# Autodesk Inventor assembly: 536206 ADN-12-15-A-P-A---(asm_0)
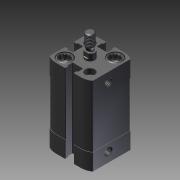
[picture p0: Inventor's stored thumbnail of the model, 180x180]
Saved by Autodesk Inventor 2011 SP1 (Build 150282100, 282)
## iProperties
Created: 2018-05-28
Part Number: 536206 ADN-12-15-A-P-A---(asm_0)
Catalog Web Link: www.cadenas.de
Description: ADN-Compact cylinder
Vendor: FESTO
Document SubType Name: Assembly
Designer: psAdmin
Manufacturer: FESTO
Mass: 95 g
Category: PARTsolutions
Company: FESTO
Title: 536206 ADN-12-15-A-P-A
Author: Cadenas PARTsolutions
Comments: Compact cylinder
PSOL_IDENT_0: {$CADENAS_DATA\23d-libs\festo\parts\a\adn\adn_std_tab.prj},213 {VTYP=3D},{STYP=ASSTAB},{NB=536206 AD
PSOL_IDENT_1: N-12-15-A-P-A---(asm_0)},{LINA=536206 ADN-12-15-A-P-A},{NN=ADN},{DATE=17.05.2018 10:40:18},{GEOMDATE=
PSOL_IDENT_2: 24.04.2017 11:47:47},{VERSION=},{LINEID=140},{LINESUBID=-1},{WBVAR=HUBST}  {NB=536206 ADN-12-15-A-P-
PSOL_IDENT_3: A---(asm_0)},{LINA=536206 ADN-12-15-A-P-A},{KT=DUMMY},{TNR=536206},{TYP=ADN-12-15-A-P-A},{KDM=12},{H
PSOL_IDENT_4: UB=15},{HUBST=0},{DF=P},{TH=A},{Q=0},{S2=0},{K2=0},{K5=0},{K8=0},{ZZ=0},{A=10.000},{AF=8.000},{BG=17
PSOL_IDENT_5: .000},{D1=9.000},{D5=6.000},{E=27.500},{EE=M5},{EEN=5.000},{EEK=4.019},{G=10.500},{KF=M3},{KFN=3.000
PSOL_IDENT_6: },{KFK=2.459},{KFNW=3},{KFKW=2.459},{KK=M5},{KKN=5.000},{KKK=4.019},{KKNW=5},{KKKW=4.019},{L3=3.500}
PSOL_IDENT_7: ,{L12=2.700},{MM=6.000},{PL=6.000},{RR=3.200},{RT=M4},{RTN=4.000},{RTK=3.242},{SW=5.000},{T1=2.100},
PSOL_IDENT_8: {T4=1.500},{TG=16.000},{WH=4.200},{ZA=35.000},{ZB=39.200},{J3=2.000},{SWQ=5.000},{RA=0.000},{RU=16.6
PSOL_IDENT_9: 00},{RT1=3.400},{RB1=5.400},{RB2=6.800},{R1=10.350},{R2=0.600},{FORM=1},{MASSBKS=0.009},{MASSHKS=0.0
PSOL_IDENT_10: 02},{MASSBZR=0.077},{MASSHZR=0.012},{CNSMASSEXACT=0.095},{PPATH=assemblies/adn_asmtpl.prj}
NN: ADN
NT: Compact cylinder
NB: 536206 ADN-12-15-A-P-A---(asm_0)
NBSYN: $TNR. $TYP.---(asm_$HUBST.)
LINA: 536206 ADN-12-15-A-P-A
OFFICIAL_STANDARD_NUMBERS: ISO 21287
TNR: 536206
TYP: ADN-12-15-A-P-A
KDM: 12
HUB: 15
HUBST: 0
DF: P
TH: A
A: 10.000
AF: 8.000
BG: 17.000
D1: 9.000
D5: 6.000
E: 27.500
EE: M5
G: 10.500
KF: M3
KK: M5
L3: 3.500
L12: 2.700
MM: 6.000
PL: 6.000
RR: 3.200
RT: M4
SW: 5.000
T1: 2.100
T4: 1.500
TG: 16.000
WH: 4.200
ZA: 35.000
ZB: 39.200
J3: 2.000
RA: 0.000
RU: 16.600
R1: 10.350
R2: 0.600
CNSMASSEXACT: 0.095
SUPPLIER: FESTO
ARTICLENO: 536206 ADN-12-15-A-P-A---(asm_0)
BOMINFO: 536206 ADN-12-15-A-P-A
CREATOR: CADENAS GmbH
## Documents named in this file (3)
- p:\temp\worker_4\2340_2584\cad_41_02018052900044819715799192d056f_000000_00_00_000001\536206 ADN-12-15-A-P-A---(asm_0).iam
- p:\temp\worker_4\2340_2584\cad_41_02018052900044819715799192d056f_000000_00_00_000001\536203 ADN-15-P---(Z).ipt
- p:\temp\worker_4\2340_2584\cad_41_02018052900044819715799192d056f_000000_00_00_000001\536203 ADN-15-P-A_(KS).ipt
## Components (2 placed, 2 different names)
1. 536203 ADN-15-P---(Z):1 — CYLINDER_Z@1 <-> PISTON_Z@2, CYLINDER_YZ@1 <-> PISTON_YZ@2
2. 536203 ADN-15-P-A_(KS):1 — CYLINDER_Z@1 <-> PISTON_Z@2, CYLINDER_YZ@1 <-> PISTON_YZ@2
## Relationships (2: Mate 1, Angle 1)
- CYLINDER_Z@1 <-> PISTON_Z@2 [Mate]: 536203 ADN-15-P---(Z):1 ↔ 536203 ADN-15-P-A_(KS):1
- CYLINDER_YZ@1 <-> PISTON_YZ@2 [Angle] (0 deg): 536203 ADN-15-P---(Z):1 ↔ 536203 ADN-15-P-A_(KS):1
